# Autodesk Inventor assembly: Сборка2
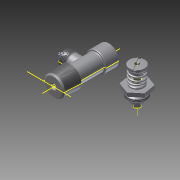
[picture p0: Inventor's stored thumbnail of the model, 180x180]
Saved by Autodesk Inventor 2012 SP2 (Build 160219200, 219)
## iProperties
Created: 2014-05-12
Part Number: Сборка2
Document SubType Name: Assembly
Designer: N750
Author: N750
## Documents named in this file (10)
- C:\Users\N750\Documents\Сборка2.iam
- J:\Сборка1\Зад22.ipt
- J:\Сборка1\Поз 9 уплотнение.ipt
- J:\Сборка1\Поз 11 Клапан.ipt
- J:\Сборка1\Поз5 Муфта.ipt
- J:\Сборка1\Поз12 Стержень.ipt
- J:\Сборка1\Поз 7 Прокладка.ipt
- J:\Сборка1\Поз 2 Гайка.ipt
- J:\Сборка1\Поз 4 Гайка.ipt
- J:\Сборка1\Поз3 Пружина.ipt
## Components (9 placed, 9 different names)
1. Зад22:1 — Совмещение:1, Совмещение:2
2. Поз 9 уплотнение:1 — Вставка:1, Совмещение:1
3. Поз 11 Клапан:1 — Вставка:1
4. Поз5 Муфта:1 — Совмещение:2
5. Поз12 Стержень:1 — Вставка:2, Вставка:4
6. Поз 7 Прокладка:1 — Вставка:2, Вставка:5
7. Поз 2 Гайка:1 — Вставка:5
8. Поз 4 Гайка:1 — Вставка:4, Совмещение:3
9. Поз3 Пружина:1 — Совмещение:3
## Relationships (7: Insert 4, Mate 3)
- Вставка:1 [Insert]: Поз 9 уплотнение:1 ↔ Поз 11 Клапан:1
- Совмещение:1 [Mate]: Зад22:1 ↔ Поз 9 уплотнение:1
- Совмещение:2 [Mate]: Зад22:1 ↔ Поз5 Муфта:1
- Вставка:2 [Insert]: Поз12 Стержень:1 ↔ Поз 7 Прокладка:1
- Вставка:4 [Insert]: Поз12 Стержень:1 ↔ Поз 4 Гайка:1
- Вставка:5 [Insert]: Поз 7 Прокладка:1 ↔ Поз 2 Гайка:1
- Совмещение:3 [Mate]: Поз 4 Гайка:1 ↔ Поз3 Пружина:1
